# Autodesk Inventor assembly: robotarm
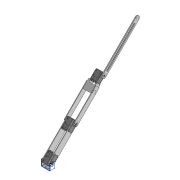
[picture p0: Inventor's stored thumbnail of the model, 180x180]
Saved by Autodesk Inventor 2020 (Build 240168000, 168)
## iProperties
Created: 2020-11-05
Part Number: robotarm
Document SubType Name: Assembly
Designer: 이호석
Mass: 696.346 g
Surface Area: 1569.88 cm^2
Volume: 456.832 cm^3
Density: 1.52429 g/cm^3
Author: 이호석
## Documents named in this file (8)
- C:\Inventor\Embedded_contest\robotarm\robotarm.iam
- C:\Inventor\Embedded_contest\ex106\EX106_H.ipt
- C:\Inventor\Embedded_contest\robotarm\bottom.ipt
- C:\Inventor\Embedded_contest\robotarm\bar1.ipt
- C:\Inventor\Embedded_contest\robotarm\bar2.ipt
- C:\Inventor\Embedded_contest\rx64\RX64_N.ipt
- C:\Inventor\Embedded_contest\robotarm\bar3.ipt
- C:\Inventor\Embedded_contest\robotarm\link.ipt
## Components (10 placed, 7 different names)
1. bottom:1 — 삽입:1, 삽입:32
2. EX106_H:1 — 삽입:1, 플러쉬:1, 플러쉬:2, 플러쉬:3, 메이트:1, 메이트:2, 삽입:3, 삽입:4, 메이트:3, 삽입:7, 삽입:8, 삽입:32
3. EX106_H:2 — 플러쉬:1, 플러쉬:2, 플러쉬:3, 메이트:1, 삽입:5, 삽입:6, 삽입:9, 삽입:10, 플러쉬:4, 플러쉬:5, 플러쉬:6, 삽입:33
4. bar1:1 — 메이트:2, 삽입:3, 삽입:4, 삽입:5, 삽입:6
5. bar1:2 — 메이트:3, 삽입:7, 삽입:8, 삽입:9, 삽입:10
6. bar2:1 — 삽입:20, 삽입:21, 삽입:22, 삽입:23
7. bar2:2 — 메이트:7, 삽입:24, 삽입:25, 삽입:26, 삽입:27, 삽입:33
8. RX64_N:1 — 플러쉬:4, 플러쉬:5, 플러쉬:6, 메이트:6, 삽입:17, 삽입:18, 삽입:19, 삽입:28, 삽입:29, 삽입:30, 삽입:31
9. bar3:1 — 메이트:6, 삽입:17, 삽입:18, 삽입:19
10. link:1 — 메이트:7, 삽입:20, 삽입:21, 삽입:22, 삽입:23, 삽입:24, 삽입:25, 삽입:26, 삽입:27, 삽입:28, 삽입:29, 삽입:30, 삽입:31
## Relationships (37: Insert 26, Flush 6, Mate 5)
- 삽입:1 [Insert]: bottom:1 ↔ EX106_H:1
- 플러쉬:1 [Flush]: EX106_H:1 ↔ EX106_H:2
- 플러쉬:2 [Flush]: EX106_H:1 ↔ EX106_H:2
- 플러쉬:3 [Flush]: EX106_H:1 ↔ EX106_H:2
- 메이트:1 [Mate] (-240 mm): EX106_H:1 ↔ EX106_H:2
- 메이트:2 [Mate]: EX106_H:1 ↔ bar1:1
- 삽입:3 [Insert]: EX106_H:1 ↔ bar1:1
- 삽입:4 [Insert]: EX106_H:1 ↔ bar1:1
- 삽입:5 [Insert]: EX106_H:2 ↔ bar1:1
- 삽입:6 [Insert]: EX106_H:2 ↔ bar1:1
- 메이트:3 [Mate]: EX106_H:1 ↔ bar1:2
- 삽입:7 [Insert]: EX106_H:1 ↔ bar1:2
- 삽입:8 [Insert]: EX106_H:1 ↔ bar1:2
- 삽입:9 [Insert]: EX106_H:2 ↔ bar1:2
- 삽입:10 [Insert]: EX106_H:2 ↔ bar1:2
- 플러쉬:4 [Flush]: EX106_H:2 ↔ RX64_N:1
- 플러쉬:5 [Flush]: EX106_H:2 ↔ RX64_N:1
- 플러쉬:6 [Flush] (250 mm): EX106_H:2 ↔ RX64_N:1
- 메이트:6 [Mate]: RX64_N:1 ↔ bar3:1
- 삽입:17 [Insert]: RX64_N:1 ↔ bar3:1
- 삽입:18 [Insert]: RX64_N:1 ↔ bar3:1
- 삽입:19 [Insert]: RX64_N:1 ↔ bar3:1
- 메이트:7 [Mate]: bar2:2 ↔ link:1
- 삽입:20 [Insert]: bar2:1 ↔ link:1
- 삽입:21 [Insert]: bar2:1 ↔ link:1
- 삽입:22 [Insert]: bar2:1 ↔ link:1
- 삽입:23 [Insert]: bar2:1 ↔ link:1
- 삽입:24 [Insert]: bar2:2 ↔ link:1
- 삽입:25 [Insert]: bar2:2 ↔ link:1
- 삽입:26 [Insert]: bar2:2 ↔ link:1
- 삽입:27 [Insert]: bar2:2 ↔ link:1
- 삽입:28 [Insert]: RX64_N:1 ↔ link:1
- 삽입:29 [Insert]: RX64_N:1 ↔ link:1
- 삽입:30 [Insert]: RX64_N:1 ↔ link:1
- 삽입:31 [Insert]: RX64_N:1 ↔ link:1
- 삽입:32 [Insert]: bottom:1 ↔ EX106_H:1
- 삽입:33 [Insert]: EX106_H:2 ↔ bar2:2
